# Autodesk Inventor assembly: baseAssembly01
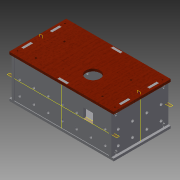
[picture p0: Inventor's stored thumbnail of the model, 180x180]
Saved by Autodesk Inventor 2013 (Build 170138000, 138)
## iProperties
Created: 2014-10-07
Part Number: baseAssembly01
Document SubType Name: Assembly
Designer: Nano
Author: Nano
## Documents named in this file (5)
- C:\Users\Nano\Documents\InventorByron\InventorMasterProject\panTiltSystem\baseAssembly01.iam
- C:\Users\Nano\Documents\InventorByron\InventorMasterProject\panTiltSystem\baseBoxShortSideRB02.ipt
- C:\Users\Nano\Documents\InventorByron\InventorMasterProject\panTiltSystem\basePanel01.ipt
- C:\Users\Nano\Documents\InventorByron\InventorMasterProject\panTiltSystem\baseBoxLongSide01.ipt
- C:\Users\Nano\Documents\InventorByron\InventorMasterProject\panTiltSystem\panStepperMountRB02.ipt
## Components (6 placed, 4 different names)
1. panStepperMountRB02:1 — Mate:1, Mate:2, Mate:3, Mate:4, Mate:5, Mate:6, Mate:7
2. baseBoxShortSideRB02:1 — Mate:1, Mate:2, Mate:3, Flush:1, Mate:8, Mate:9
3. baseBoxShortSideRB02:2 — Mate:4, Mate:5, Mate:6, Flush:2
4. basePanel01:1 — Flush:1
5. baseBoxLongSide01:1 — Flush:2
6. baseBoxLongSide01:2 — Mate:7, Mate:8, Mate:9
## Relationships (11: Mate 9, Flush 2)
- Mate:1: panStepperMountRB02:1 ↔ baseBoxShortSideRB02:1
- Mate:2: panStepperMountRB02:1 ↔ baseBoxShortSideRB02:1
- Mate:3: panStepperMountRB02:1 ↔ baseBoxShortSideRB02:1
- Mate:4: panStepperMountRB02:1 ↔ baseBoxShortSideRB02:2
- Mate:5: panStepperMountRB02:1 ↔ baseBoxShortSideRB02:2
- Mate:6: panStepperMountRB02:1 ↔ baseBoxShortSideRB02:2
- Flush:1: baseBoxShortSideRB02:1 ↔ basePanel01:1
- Flush:2 (-1.5875 mm): baseBoxShortSideRB02:2 ↔ baseBoxLongSide01:1
- Mate:7: panStepperMountRB02:1 ↔ baseBoxLongSide01:2
- Mate:8: baseBoxShortSideRB02:1 ↔ baseBoxLongSide01:2
- Mate:9: baseBoxShortSideRB02:1 ↔ baseBoxLongSide01:2
